# Autodesk Inventor assembly: GFRP_T2_11
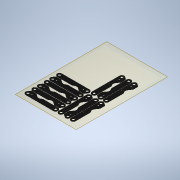
[picture p0: Inventor's stored thumbnail of the model, 180x180]
Saved by Autodesk Inventor 2020 (Build 240168000, 168)
## iProperties
Created: 2021-08-27
Part Number: GFRP_T2_11
Document SubType Name: Assembly
Designer: Masato
Author: Masato
## Documents named in this file (3)
- C:\Inventor\SUSTAINA-OP\Cam\GFRP_T2_11.iam
- C:\Inventor\SUSTAINA-OP\Cam\DisposableBoard.ipt
- C:\Inventor\SUSTAINA-OP\LowerBody\Link\BackLink_frame.ipt
## Components (13 placed, 2 different names)
1. DisposableBoard:1 — メイト:2, メイト:1, フラッシュ:1, フラッシュ:2, メイト:4, メイト:5, フラッシュ:3, 正接:1, 正接:2, 角度:1, メイト:7, 正接:3, メイト:8, 正接:5
2. BackLink_frame:1 — メイト:4, メイト:6, 正接:2
3. BackLink_frame:2 — メイト:5, フラッシュ:3, メイト:6, 正接:1, 正接:4
4. BackLink_frame:4
5. BackLink_frame:5
6. BackLink_frame:6
7. BackLink_frame:7
8. BackLink_frame:9 — メイト:8, メイト:9, 正接:5
9. BackLink_frame:11
10. BackLink_frame:8 — 角度:1, メイト:7, 正接:3, 正接:4, メイト:9
11. BackLink_frame:10
12. BackLink_frame:12
13. BackLink_frame:13
## Component patterns: (3 elements, first: BackLink_frame:1 + BackLink_frame:2), (2 elements, first: BackLink_frame:9), (2 elements, first: BackLink_frame:8), コンポーネント パターン 5:2 (2 elements)
## Relationships (17: Mate 8, Tangent 5, Flush 3, Angle 1)
- メイト:2 [Mate]: DisposableBoard:1
- メイト:1 [Mate]: DisposableBoard:1
- フラッシュ:1 [Flush]: DisposableBoard:1
- フラッシュ:2 [Flush]: DisposableBoard:1
- メイト:4 [Mate]: DisposableBoard:1 ↔ BackLink_frame:1
- メイト:5 [Mate]: DisposableBoard:1 ↔ BackLink_frame:2
- フラッシュ:3 [Flush] (2 mm): DisposableBoard:1 ↔ BackLink_frame:2
- メイト:6 [Mate] (2.5 mm): BackLink_frame:1 ↔ BackLink_frame:2
- 正接:1 [Tangent] (2 mm): DisposableBoard:1 ↔ BackLink_frame:2
- 正接:2 [Tangent] (2 mm): DisposableBoard:1 ↔ BackLink_frame:1
- 角度:1 [Angle] (0 deg): DisposableBoard:1 ↔ BackLink_frame:8
- メイト:7 [Mate]: DisposableBoard:1 ↔ BackLink_frame:8
- 正接:3 [Tangent] (2 mm): DisposableBoard:1 ↔ BackLink_frame:8
- 正接:4 [Tangent] (2.5 mm): BackLink_frame:2 ↔ BackLink_frame:8
- メイト:8 [Mate]: DisposableBoard:1 ↔ BackLink_frame:9
- メイト:9 [Mate] (2.5 mm): BackLink_frame:9 ↔ BackLink_frame:8
- 正接:5 [Tangent] (2 mm): DisposableBoard:1 ↔ BackLink_frame:9
